# Autodesk Inventor assembly: 95652
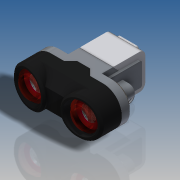
[picture p0: Inventor's stored thumbnail of the model, 180x180]
Saved by Autodesk Inventor 2016 SP2 (Build 200236200, 236)
## iProperties
Created: 2015-08-26
Part Number: 95652
Document SubType Name: Assembly
Designer: D. Kohfeld
Mass: 31.0872 g
Surface Area: 298.383 cm^2
Volume: 18.1688 cm^3
Density: 1.71102 g/cm^3
Author: D. Kohfeld
## Documents named in this file (9)
- A:\LEGO Pieces\EV3\95652.iam
- A:\LEGO Pieces\EV3\99378-LtBluishGray.ipt
- A:\LEGO Pieces\EV3\99376-White.ipt
- A:\LEGO Pieces\EV3\54732b-LtBluishGray.ipt
- A:\LEGO Pieces\EV3\99401-RedRubber.ipt
- A:\LEGO Pieces\EV3\99957-ElectricAlloy.ipt
- A:\LEGO Pieces\EV3\10361-TransRed.ipt
- A:\LEGO Pieces\EV3\99390-Black.ipt
- A:\LEGO Pieces\EV3\99391-LtBluishGray.ipt
## Components (10 placed, 8 different names)
1. 99378-LtBluishGray:1 — Flush:1, Flush:2, Mate:1, Mate:3, Flush:4, Flush:5, Flush:6, Mate:4, Flush:7, Mate:5, Mate:6
2. 99376-White:1 — Flush:1, Flush:2, Mate:1, Mate:2, Flush:3
3. 54732b-LtBluishGray:1 — Mate:2, Mate:3, Flush:3
4. 99401-RedRubber:1 — Insert:1, Insert:3, Mate:8
5. 99401-RedRubber:2 — Insert:2, Insert:4
6. 99957-ElectricAlloy:1 — Insert:1
7. 99957-ElectricAlloy:2 — Insert:2
8. 10361-TransRed:1 — Flush:4, Insert:3, Insert:4, Mate:7
9. 99390-Black:1 — Flush:5, Flush:6, Mate:4
10. 99391-LtBluishGray:1 — Flush:7, Mate:5, Mate:6, Mate:7, Mate:8
## Relationships (19: Mate 8, Flush 7, Insert 4)
- Insert:1: 99401-RedRubber:1 ↔ 99957-ElectricAlloy:1
- Insert:2: 99401-RedRubber:2 ↔ 99957-ElectricAlloy:2
- Flush:1: 99378-LtBluishGray:1 ↔ 99376-White:1
- Flush:2: 99378-LtBluishGray:1 ↔ 99376-White:1
- Mate:1: 99378-LtBluishGray:1 ↔ 99376-White:1
- Mate:2: 99376-White:1 ↔ 54732b-LtBluishGray:1
- Mate:3: 99378-LtBluishGray:1 ↔ 54732b-LtBluishGray:1
- Flush:3: 99376-White:1 ↔ 54732b-LtBluishGray:1
- Flush:4: 99378-LtBluishGray:1 ↔ 10361-TransRed:1
- Flush:5: 99378-LtBluishGray:1 ↔ 99390-Black:1
- Flush:6: 99378-LtBluishGray:1 ↔ 99390-Black:1
- Mate:4: 99378-LtBluishGray:1 ↔ 99390-Black:1
- Insert:3: 99401-RedRubber:1 ↔ 10361-TransRed:1
- Insert:4: 99401-RedRubber:2 ↔ 10361-TransRed:1
- Flush:7: 99378-LtBluishGray:1 ↔ 99391-LtBluishGray:1
- Mate:5: 99378-LtBluishGray:1 ↔ 99391-LtBluishGray:1
- Mate:6: 99378-LtBluishGray:1 ↔ 99391-LtBluishGray:1
- Mate:7: 10361-TransRed:1 ↔ 99391-LtBluishGray:1
- Mate:8: 99401-RedRubber:1 ↔ 99391-LtBluishGray:1
